# Autodesk Inventor assembly: Air Heater Controller
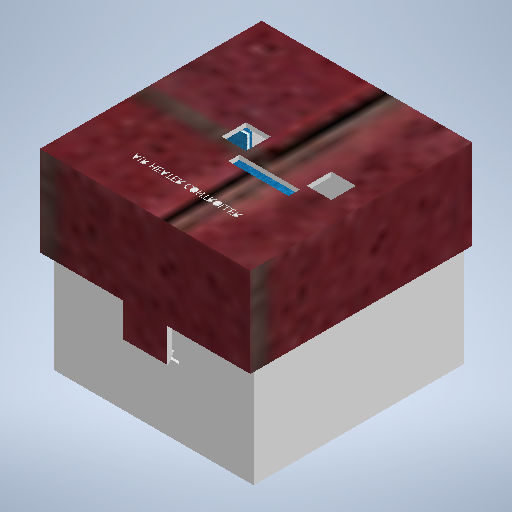
[picture p0: Inventor's stored thumbnail of the model, 512x512]
Saved by Autodesk Inventor 2025.2 (Build 292293000, 293)
## iProperties
Created: 2025-09-19
Part Number: Air Heater Controller
Document SubType Name: Assembly
Designer: TSO
Author: TSO
## Documents named in this file (4)
- H:\Skole\IIA3220\Hardware\Air Heater Controller.iam
- H:\Skole\IIA3220\Hardware\Arduino_case.ipt
- H:\Skole\IIA3220\Hardware\Breadboard_insert.ipt
- H:\Skole\IIA3220\Hardware\Arduino_case_lid_MIR.ipt
## Components (3 placed, 3 different names)
1. Arduino_case:1 — Rigid:1, Rigid:2
2. Breadboard_insert:1 — Rigid:1
3. Arduino_case_lid_MIR:1 — Rigid:2
## Relationships (2: WeldJoint 2)
- Rigid:1 [WeldJoint]: Arduino_case:1 ↔ Breadboard_insert:1
- Rigid:2 [WeldJoint]: Arduino_case:1 ↔ Arduino_case_lid_MIR:1
## Named parameters: Finish1_Area = 183.509, Finish2_Area = 249.109
note: some values were not read from the file. Shown as the stored number, unit unknown: "Finish1_Area", "Finish2_Area".
